# Autodesk Inventor assembly: wheel_axle_assembly
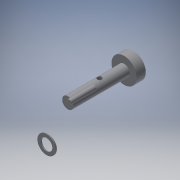
[picture p0: Inventor's stored thumbnail of the model, 180x180]
Saved by Autodesk Inventor 2018 (Build 220112000, 112)
## iProperties
Created: 2018-04-03
Part Number: wheel_axle_assembly
Document SubType Name: Assembly
Designer: dvyen
Author: dvyen
## Documents named in this file (6)
- C:\Users\dvyen\source\repos\micromouse-2\drivetrain\wheel_axle_assembly.iam
- C:\Users\dvyen\source\repos\micromouse-2\drivetrain\axle_TX2437.ipt
- C:\Users\dvyen\source\repos\micromouse-2\drivetrain\bushing_TX1675.ipt
- C:\Users\dvyen\source\repos\micromouse-2\drivetrain\pin_AX31028.ipt
- C:\Users\dvyen\source\repos\micromouse-2\drivetrain\ptfe_washer_TX1985.ipt
- C:\Users\dvyen\source\repos\micromouse-2\drivetrain\ptfe_washer_TX1985_CPY.ipt
## Components (5 placed, 5 different names)
1. axle_TX2437:1 — Insert:1
2. bushing_TX1675:1 — Insert:1
3. pin_AX31028:1
4. ptfe_washer_TX1985:1
5. ptfe_washer_TX1985_CPY:1
## Relationships (1: Insert 1)
- Insert:1: axle_TX2437:1 ↔ bushing_TX1675:1
